# Autodesk Inventor assembly: Bot 1
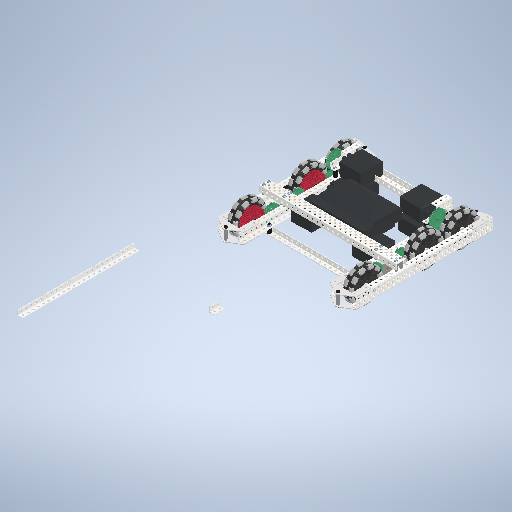
[picture p0: Inventor's stored thumbnail of the model, 512x512]
Saved by Autodesk Inventor 2025.2 (Build 292293000, 293)
## iProperties
Created: 2025-03-17
Part Number: Bot 1
Document SubType Name: Assembly
Designer: Jahan
Author: Jahan
## Documents named in this file (43)
- C:\1629X-7700R-Worlds-Bot\Bot 1\Bot 1.iam
- C:\1629X-7700R-Worlds-Bot\VEX-CAD-Inventor-1.4.2\Structure\C Channel\Aluminum 1x2x1\Alu C 1x2x1x27.ipt
- C:\1629X-7700R-Worlds-Bot\VEX-CAD-Inventor-1.4.2\Structure\C Channel\Aluminum 1x2x1\Alu C 1x2x1x19.ipt
- C:\1629X-7700R-Worlds-Bot\VEX-CAD-Inventor-1.4.2\Motion\Gears\HS Gear.iam
- C:\1629X-7700R-Worlds-Bot\VEX-CAD-Inventor-1.4.2\Motion\Wheels\Omni Wheel\3.25 Omni AS, No Insert.iam
- C:\1629X-7700R-Worlds-Bot\VEX-CAD-Inventor-1.4.2\Motion\Wheels\Omni Wheel.iam
- C:\1629X-7700R-Worlds-Bot\VEX-CAD-Inventor-1.4.2\Motion\Gears\HS Gear\HS 48T Gear, Circle.iam
- C:\1629X-7700R-Worlds-Bot\VEX-CAD-Inventor-1.4.2\Structure\Standoff.ipt
- C:\1629X-7700R-Worlds-Bot\VEX-CAD-Inventor-1.4.2\Structure\Standoff\Standoff .50.ipt
- C:\1629X-7700R-Worlds-Bot\VEX-CAD-Inventor-1.4.2\Motion\Spacers\Washer Teflon.ipt
- C:\1629X-7700R-Worlds-Bot\VEX-CAD-Inventor-1.4.2\Motion\Spacers\Spacer Nylon .375 OD\NSpacer .375 OD x .125.ipt
- C:\1629X-7700R-Worlds-Bot\VEX-CAD-Inventor-1.4.2\Motion\Spacers\Spacer Nylon .375 OD.ipt
- C:\1629X-7700R-Worlds-Bot\VEX-CAD-Inventor-1.4.2\Motion\Spacers\Washer Teflon\TWasher .375 OD x .06250.ipt
- C:\1629X-7700R-Worlds-Bot\VEX-CAD-Inventor-1.4.2\Structure\Hardware\alu_nylock.ipt
- C:\1629X-7700R-Worlds-Bot\VEX-CAD-Inventor-1.4.2\Motion\Gears\LS 36T Gear.ipt
- C:\1629X-7700R-Worlds-Bot\VEX-CAD-Inventor-1.4.2\Motion\Gears\HS Gear\24T HS Gear Cut.iam
- C:\1629X-7700R-Worlds-Bot\VEX-CAD-Inventor-1.4.2\Motion\Shaft LS\Bearing Flat Low Profile.ipt
- C:\1629X-7700R-Worlds-Bot\VEX-CAD-Inventor-1.4.2\Structure\Hardware\Screw Steel - Hex.ipt
- C:\1629X-7700R-Worlds-Bot\VEX-CAD-Inventor-1.4.2\Structure\Hardware\Screw Steel - Hex\SScrew Hex Smooth 1.750.ipt
- C:\1629X-7700R-Worlds-Bot\VEX-CAD-Inventor-1.4.2\Structure\C Channel\Aluminum 1x2x1\Alu C 1x2x1x26.ipt
- C:\1629X-7700R-Worlds-Bot\VEX-CAD-Inventor-1.4.2\Structure\Hardware\Screw Aluminum - Flat Head\AScrew Flat Head Threaded .250.ipt
- C:\1629X-7700R-Worlds-Bot\VEX-CAD-Inventor-1.4.2\Motion\Spacers\Spacer Nylon .375 OD\NSpacer .375 OD x .250.ipt
- C:\1629X-7700R-Worlds-Bot\VEX-CAD-Inventor-1.4.2\Structure\Standoff\Standoff .75.ipt
- C:\1629X-7700R-Worlds-Bot\VEX-CAD-Inventor-1.4.2\Structure\Hardware\Nut Thin Nylock.ipt
- C:\1629X-7700R-Worlds-Bot\VEX-CAD-Inventor-1.4.2\Structure\Hardware\Screw Steel - Star\SScrew Star Smooth .250.ipt
- C:\1629X-7700R-Worlds-Bot\VEX-CAD-Inventor-1.4.2\Structure\Hardware\Screw Steel - Star.ipt
- C:\1629X-7700R-Worlds-Bot\Bot 1\Plastic\backFunnel.ipt
- C:\1629X-7700R-Worlds-Bot\VEX-CAD-Inventor-1.4.2\Structure\Standoff\Standoff 1.00.ipt
- C:\1629X-7700R-Worlds-Bot\VEX-CAD-Inventor-1.4.2\Structure\Angle\Aluminum 1x1\Alu Angle 1x1x19.ipt
- C:\1629X-7700R-Worlds-Bot\VEX-CAD-Inventor-1.4.2\Motion\Spacers\Spacer Nylon .375 OD\NSpacer .375 OD x .500.ipt
- C:\1629X-7700R-Worlds-Bot\VEX-CAD-Inventor-1.4.2\Structure\Hardware\Screw Steel - Star\SScrew Star Smooth .500.ipt
- C:\1629X-7700R-Worlds-Bot\VEX-CAD-Inventor-1.4.2\Electronics\V5 Simple Motor.ipt
- C:\1629X-7700R-Worlds-Bot\VEX-CAD-Inventor-1.4.2\Structure\Hardware\Screw Steel - Star\SScrew Star Smooth .750.ipt
- C:\1629X-7700R-Worlds-Bot\VEX-CAD-Inventor-1.4.2\Structure\Hardware\Screw Nylon - Flat Head\NScrew Flat Head Threaded .250.ipt
- C:\1629X-7700R-Worlds-Bot\VEX-CAD-Inventor-1.4.2\Electronics\V5 Simple Brain.ipt
- C:\1629X-7700R-Worlds-Bot\Bot 1\Plastic\frontFunnel.ipt
- C:\1629X-7700R-Worlds-Bot\VEX-CAD-Inventor-1.4.2\Structure\Angle\Aluminum 1x1\Alu Angle 1x1x2.ipt
- C:\1629X-7700R-Worlds-Bot\VEX-CAD-Inventor-1.4.2\Structure\Angle\Aluminum 1x1\Alu Angle 1x1x23.ipt
- C:\1629X-7700R-Worlds-Bot\VEX-CAD-Inventor-1.4.2\Structure\C Channel\Aluminum 1x2x1\Alu C 1x2x1x3.ipt
- C:\1629X-7700R-Worlds-Bot\VEX-CAD-Inventor-1.4.2\Motion\Spacers\Spacer Nylon .375 OD\NSpacer .375 OD x .375.ipt
- C:\1629X-7700R-Worlds-Bot\VEX-CAD-Inventor-1.4.2\Structure\Angle\Aluminum 1x1\Alu Angle 1x1x5.ipt
- C:\1629X-7700R-Worlds-Bot\VEX-CAD-Inventor-1.4.2\Structure\Hardware\Screw Steel - Star\SScrew Star Smooth 1.000.ipt
- C:\1629X-7700R-Worlds-Bot\VEX-CAD-Inventor-1.4.2\Structure\Hardware\Screw Steel - Star\SScrew Star Smooth .625.ipt
## Components (175 placed, 35 different names)
1. Alu C 1x2x1x26:2 — Insert:72, Insert:73, Insert:74, Insert:105, Insert:106, Insert:130, Insert:132, Insert:141, Insert:142, Insert:143, Insert:144, Insert:151, Insert:152, Insert:163, Mate:8, Flush:1, Insert:164, Insert:165, Insert:169, Insert:181, Insert:186, Insert:206, Insert:210, Insert:213, Insert:228, Insert:229, Insert:257, Insert:264, Insert:274, Insert:275, Insert:276
2. Alu C 1x2x1x26:1 — Insert:5, Insert:6, Insert:75, Insert:76, Insert:77, Insert:107, Insert:108, Insert:125, Insert:126, Insert:139, Insert:140, Insert:145, Insert:146, Insert:147, Insert:148, Insert:149, Insert:150, Insert:182, Insert:184, Insert:204, Insert:211, Insert:212, Insert:225, Insert:227, Insert:233, Insert:241, Insert:242, Insert:243, Insert:252
3. Alu C 1x2x1x27:3 — Insert:5, Insert:6, Insert:7, Insert:8, Insert:9, Insert:10
4. Alu C 1x2x1x27:4 — Insert:7, Insert:8, Insert:52, Insert:58, Insert:65, Insert:81, Insert:82, Insert:83, Insert:127, Insert:128, Insert:170, Insert:171, Insert:172, Insert:173, Insert:183, Insert:203
5. Alu C 1x2x1x27:5 — Insert:9, Insert:10, Insert:25, Insert:31, Insert:39, Insert:43, Insert:44, Insert:45, Insert:46, Insert:78, Insert:79, Insert:80, Insert:129, Insert:131, Insert:166, Insert:167, Insert:168, Insert:180, Insert:205, Insert:208, Insert:209
6. HS 48T Gear, Circle:3 [sub-assembly] — Mate:1
7. 3.25 Omni AS, No Insert:4 [sub-assembly] — Mate:1
8. NSpacer .375 OD x .125:2
9. TWasher .375 OD x .06250:2 — Insert:23
10. alu_nylock:3 — Insert:23, Insert:24
11. Standoff .50:3 — Insert:24, Insert:25
12. HS 48T Gear, Circle:4 [sub-assembly] — Mate:2
13. 3.25 Omni AS, No Insert:5 [sub-assembly] — Mate:2
14. NSpacer .375 OD x .125:3
15. TWasher .375 OD x .06250:3
16. alu_nylock:4
17. Standoff .50:4 — Insert:31
18. HS 48T Gear, Circle:5 [sub-assembly] — Mate:3
19. 3.25 Omni AS, No Insert:6 [sub-assembly] — Mate:3
20. NSpacer .375 OD x .125:4
21. TWasher .375 OD x .06250:4
22. alu_nylock:5
23. Standoff .50:5 — Insert:39
24. Bearing Flat Low Profile:1 — Insert:43, Insert:44
25. Bearing Flat Low Profile:2 — Insert:45, Insert:46
26. HS 48T Gear, Circle:6 [sub-assembly]
27. 3.25 Omni AS, No Insert:7 [sub-assembly]
28. NSpacer .375 OD x .125:6
29. TWasher .375 OD x .06250:5
30. alu_nylock:6
31. Standoff .50:6 — Insert:52
32. HS 48T Gear, Circle:7 [sub-assembly]
33. 3.25 Omni AS, No Insert:8 [sub-assembly]
34. NSpacer .375 OD x .125:7
35. TWasher .375 OD x .06250:6
36. alu_nylock:7
37. Standoff .50:7 — Insert:58
38. HS 48T Gear, Circle:8 [sub-assembly]
39. 3.25 Omni AS, No Insert:9 [sub-assembly]
40. NSpacer .375 OD x .125:8
41. TWasher .375 OD x .06250:7
42. alu_nylock:8
43. Standoff .50:8 — Insert:65
44. SScrew Hex Smooth 1.750:1 — Insert:72
45. SScrew Hex Smooth 1.750:2 — Insert:74
46. SScrew Hex Smooth 1.750:3 — Insert:73
47. SScrew Hex Smooth 1.750:4 — Insert:77
48. SScrew Hex Smooth 1.750:5 — Insert:76
49. SScrew Hex Smooth 1.750:6 — Insert:75
50. AScrew Flat Head Threaded .250:1 — Insert:78
51. AScrew Flat Head Threaded .250:2 — Insert:79
52. AScrew Flat Head Threaded .250:3 — Insert:80
53. AScrew Flat Head Threaded .250:4 — Insert:81
54. AScrew Flat Head Threaded .250:5 — Insert:82
55. AScrew Flat Head Threaded .250:6 — Insert:83
56. Alu C 1x2x1x19:1 — Insert:226, Insert:230, Insert:231, Insert:253, Insert:254, Insert:258
57. Nut Thin Nylock:1 — Insert:105
58. Nut Thin Nylock:2 — Insert:108
59. Nut Thin Nylock:3 — Insert:106
60. Nut Thin Nylock:4 — Insert:107
61. backFunnel:1 — Insert:125, Insert:127, Insert:159
62. backFunnel:2 — Insert:126, Insert:128, Insert:133, Insert:160
63. backFunnel:3 — Insert:129, Insert:130, Insert:161
64. backFunnel:4 — Insert:131, Insert:132, Insert:134, Insert:162
65. Standoff 1.00:17 — Insert:134
66. Standoff 1.00:18 — Insert:133
67. SScrew Star Smooth .500:17 — Insert:141
68. SScrew Star Smooth .500:18 — Insert:146
69. SScrew Star Smooth .500:19 — Insert:144
70. SScrew Star Smooth .500:20 — Insert:145
71. SScrew Star Smooth .500:21 — Insert:143
72. SScrew Star Smooth .500:22 — Insert:139
73. SScrew Star Smooth .500:23 — Insert:140
74. SScrew Star Smooth .500:24 — Insert:142
75. V5 Simple Motor:1 — Insert:147, Insert:148
76. V5 Simple Motor:2 — Insert:149, Insert:150
77. V5 Simple Motor:4 — Insert:151, Insert:152
78. SScrew Star Smooth .750:26 — Insert:189
79. NScrew Flat Head Threaded .250:1 — Insert:159
80. NScrew Flat Head Threaded .250:2 — Insert:160
81. NScrew Flat Head Threaded .250:3 — Insert:162
82. NScrew Flat Head Threaded .250:4 — Insert:161
83. V5 Simple Motor:5 — Insert:163, Mate:8
84. V5 Simple Brain:1
85. frontFunnel:1 — Insert:164, Insert:165, Insert:166, Insert:167, Insert:177
86. frontFunnel:2 — Insert:168, Insert:169, Insert:178, Insert:179
87. frontFunnel:3 — Insert:170, Insert:171, Insert:175
88. frontFunnel:4 — Insert:172, Insert:173, Insert:174, Insert:176
89. Standoff 1.00:19 — Insert:179
90. NScrew Flat Head Threaded .250:5 — Insert:177
91. NScrew Flat Head Threaded .250:6 — Insert:178
92. Standoff 1.00:20 — Insert:176
93. NScrew Flat Head Threaded .250:7 — Insert:174
94. NScrew Flat Head Threaded .250:8 — Insert:175
95. Standoff .75:22 — Mate:16, Insert:209
96. SScrew Star Smooth .250:27 — Mate:14
97. SScrew Star Smooth .250:28 — Mate:15
98. SScrew Star Smooth .250:29 — Mate:12
99. SScrew Star Smooth .250:30 — Mate:11
100. Standoff .75:23 — Mate:10
101. Standoff .75:24 — Mate:9
102. Standoff .75:25 — Insert:197
103. Standoff .75:26 — Insert:196
104. Standoff .75:27 — Insert:193
105. Standoff .75:28 — Insert:192
106. Alu C 1x2x1x27:6 — Insert:192, Insert:193, Insert:194, Insert:195, Insert:196, Insert:197, Insert:198, Insert:199, Mate:9, Mate:10, Mate:11, Mate:12, Mate:14, Mate:15, Mate:16, Insert:207
107. SScrew Star Smooth .250:31 — Insert:198
108. SScrew Star Smooth .250:32 — Insert:199
109. SScrew Star Smooth .250:33 — Insert:195
110. SScrew Star Smooth .250:34 — Insert:194
111. SScrew Star Smooth .250:35 — Insert:181
112. SScrew Star Smooth .250:36 — Insert:180
113. SScrew Star Smooth .250:37 — Insert:182
114. SScrew Star Smooth .250:39 — Insert:183
115. NSpacer .375 OD x .125:16 — Insert:184, Insert:185
116. 24T HS Gear Cut:6 [sub-assembly] — Insert:185
117. 24T HS Gear Cut:7 [sub-assembly] — Insert:187
118. NSpacer .375 OD x .125:17 — Insert:186, Insert:187
119. Nut Thin Nylock:6 — Insert:212
120. NSpacer .375 OD x .500:18 — Insert:190, Insert:211
121. Alu Angle 1x1x19:1 — Insert:188, Insert:189, Insert:190, Insert:191
122. NSpacer .375 OD x .500:19 — Insert:191, Insert:210
123. SScrew Star Smooth .750:40 — Insert:188
124. Alu Angle 1x1x2:1
125. Alu Angle 1x1x23:1
126. SScrew Star Smooth .250:41 — Insert:203
127. SScrew Star Smooth .250:42 — Insert:204
128. Standoff .75:29 — Insert:207, Insert:208
129. SScrew Star Smooth .250:43 — Insert:206
130. SScrew Star Smooth .250:44 — Insert:205
131. Nut Thin Nylock:7 — Insert:213
132. NSpacer .375 OD x .250:22 — Insert:225, Insert:226
133. NSpacer .375 OD x .250:23 — Insert:228, Insert:230
134. NSpacer .375 OD x .250:24 — Insert:227
135. NSpacer .375 OD x .250:25 — Insert:229
136. NSpacer .375 OD x .375:26 — Insert:231, Insert:236
137. NSpacer .375 OD x .375:28 — Insert:234, Insert:235
138. NSpacer .375 OD x .250:29 — Insert:235
139. TWasher .375 OD x .06250:8 — Insert:233, Insert:234
140. LS 36T Gear:9 — Insert:238
141. Alu Angle 1x1x5:1 — Insert:236, Insert:237, Insert:239, Insert:240, Insert:247, Insert:248, Insert:251
142. TWasher .375 OD x .06250:9 — Insert:237, Insert:238
143. SScrew Star Smooth .500:45 — Insert:240
144. SScrew Star Smooth .500:46 — Insert:239
145. LS 36T Gear:10 — Insert:246
146. LS 36T Gear:11 — Insert:245
147. LS 36T Gear:12 — Insert:244
148. TWasher .375 OD x .06250:10 — Insert:241, Insert:244
149. TWasher .375 OD x .06250:11 — Insert:243, Insert:246
150. TWasher .375 OD x .06250:12 — Insert:242, Insert:245
151. V5 Simple Motor:7 — Insert:249, Insert:250
152. Alu C 1x2x1x3:1 — Insert:247, Insert:248, Insert:249, Insert:250
153. SScrew Star Smooth 1.000:49 — Insert:251
154. Nut Thin Nylock:8 — Insert:252
155. SScrew Star Smooth .625:52 — Insert:253
156. SScrew Star Smooth .625:53 — Insert:254
157. NSpacer .375 OD x .375:30
158. NSpacer .375 OD x .250:31 — Insert:259
159. TWasher .375 OD x .06250:13 — Insert:257
160. NSpacer .375 OD x .375:32 — Insert:258, Insert:260
161. V5 Simple Motor:8 — Insert:265, Insert:266
162. Alu C 1x2x1x3:2 — Insert:261, Insert:262, Insert:265, Insert:266
163. Alu Angle 1x1x5:2 — Insert:259, Insert:260, Insert:261, Insert:262, Insert:263, Insert:268, Insert:269, Insert:270
164. SScrew Star Smooth 1.000:54 — Insert:263
165. Nut Thin Nylock:9 — Insert:264
166. LS 36T Gear:13
167. TWasher .375 OD x .06250:14 — Insert:268
168. SScrew Star Smooth .500:55 — Insert:269
169. SScrew Star Smooth .500:56 — Insert:270
170. LS 36T Gear:14
171. TWasher .375 OD x .06250:15 — Insert:275
172. LS 36T Gear:15
173. TWasher .375 OD x .06250:16 — Insert:276
174. LS 36T Gear:16
175. TWasher .375 OD x .06250:17 — Insert:274
## Relationships (204: Insert 189, Mate 14, Flush 1)
- Insert:5: Alu C 1x2x1x26:1 ↔ Alu C 1x2x1x27:3
- Insert:6: Alu C 1x2x1x26:1 ↔ Alu C 1x2x1x27:3
- Insert:7: Alu C 1x2x1x27:3 ↔ Alu C 1x2x1x27:4
- Insert:8: Alu C 1x2x1x27:3 ↔ Alu C 1x2x1x27:4
- Insert:9: Alu C 1x2x1x27:3 ↔ Alu C 1x2x1x27:5
- Insert:10: Alu C 1x2x1x27:3 ↔ Alu C 1x2x1x27:5
- [Insert]: HS 48T Gear, Circle:3 ↔ 3.25 Omni AS, No Insert:4
- [Insert]: HS 48T Gear, Circle:3 ↔ NSpacer .375 OD x .125:2
- [Insert]: 3.25 Omni AS, No Insert:4 ↔ TWasher .375 OD x .06250:2
- Insert:23: TWasher .375 OD x .06250:2 ↔ alu_nylock:3
- Insert:24: alu_nylock:3 ↔ Standoff .50:3
- Insert:25: Alu C 1x2x1x27:5 ↔ Standoff .50:3
- [Insert]: HS 48T Gear, Circle:4 ↔ 3.25 Omni AS, No Insert:5
- [Insert]: HS 48T Gear, Circle:4 ↔ NSpacer .375 OD x .125:3
- [Insert]: 3.25 Omni AS, No Insert:5 ↔ TWasher .375 OD x .06250:3
- [Insert]: TWasher .375 OD x .06250:3 ↔ alu_nylock:4
- [Insert]: alu_nylock:4 ↔ Standoff .50:4
- Insert:31: Alu C 1x2x1x27:5 ↔ Standoff .50:4
- [Insert]: HS 48T Gear, Circle:5 ↔ 3.25 Omni AS, No Insert:6
- [Insert]: HS 48T Gear, Circle:5 ↔ NSpacer .375 OD x .125:4
- [Insert]: 3.25 Omni AS, No Insert:6 ↔ TWasher .375 OD x .06250:4
- [Insert]: TWasher .375 OD x .06250:4 ↔ alu_nylock:5
- [Insert]: alu_nylock:5 ↔ Standoff .50:5
- Insert:39: Alu C 1x2x1x27:5 ↔ Standoff .50:5
- Mate:1: HS 48T Gear, Circle:3 ↔ 3.25 Omni AS, No Insert:4
- Mate:2: HS 48T Gear, Circle:4 ↔ 3.25 Omni AS, No Insert:5
- Mate:3: HS 48T Gear, Circle:5 ↔ 3.25 Omni AS, No Insert:6
- Insert:43: Alu C 1x2x1x27:5 ↔ Bearing Flat Low Profile:1
- Insert:44: Alu C 1x2x1x27:5 ↔ Bearing Flat Low Profile:1
- Insert:45: Alu C 1x2x1x27:5 ↔ Bearing Flat Low Profile:2
- Insert:46: Alu C 1x2x1x27:5 ↔ Bearing Flat Low Profile:2
- [Insert]: HS 48T Gear, Circle:6 ↔ 3.25 Omni AS, No Insert:7
- [Insert]: HS 48T Gear, Circle:6 ↔ NSpacer .375 OD x .125:6
- [Insert]: 3.25 Omni AS, No Insert:7 ↔ TWasher .375 OD x .06250:5
- [Insert]: TWasher .375 OD x .06250:5 ↔ alu_nylock:6
- [Insert]: alu_nylock:6 ↔ Standoff .50:6
- [Mate]: HS 48T Gear, Circle:6 ↔ 3.25 Omni AS, No Insert:7
- Insert:52: Alu C 1x2x1x27:4 ↔ Standoff .50:6
- [Insert]: HS 48T Gear, Circle:7 ↔ 3.25 Omni AS, No Insert:8
- [Insert]: HS 48T Gear, Circle:7 ↔ NSpacer .375 OD x .125:7
- [Insert]: 3.25 Omni AS, No Insert:8 ↔ TWasher .375 OD x .06250:6
- [Insert]: TWasher .375 OD x .06250:6 ↔ alu_nylock:7
- [Insert]: alu_nylock:7 ↔ Standoff .50:7
- [Mate]: HS 48T Gear, Circle:7 ↔ 3.25 Omni AS, No Insert:8
- Insert:58: Alu C 1x2x1x27:4 ↔ Standoff .50:7
- [Insert]: HS 48T Gear, Circle:8 ↔ 3.25 Omni AS, No Insert:9
- [Insert]: HS 48T Gear, Circle:8 ↔ NSpacer .375 OD x .125:8
- [Insert]: 3.25 Omni AS, No Insert:9 ↔ TWasher .375 OD x .06250:7
- [Insert]: TWasher .375 OD x .06250:7 ↔ alu_nylock:8
- [Insert]: alu_nylock:8 ↔ Standoff .50:8
- [Mate]: HS 48T Gear, Circle:8 ↔ 3.25 Omni AS, No Insert:9
- Insert:65: Alu C 1x2x1x27:4 ↔ Standoff .50:8
- Insert:72: Alu C 1x2x1x26:2 ↔ SScrew Hex Smooth 1.750:1
- Insert:73: Alu C 1x2x1x26:2 ↔ SScrew Hex Smooth 1.750:3
- Insert:74: Alu C 1x2x1x26:2 ↔ SScrew Hex Smooth 1.750:2
- Insert:75: Alu C 1x2x1x26:1 ↔ SScrew Hex Smooth 1.750:6
- Insert:76: Alu C 1x2x1x26:1 ↔ SScrew Hex Smooth 1.750:5
- Insert:77: Alu C 1x2x1x26:1 ↔ SScrew Hex Smooth 1.750:4
- Insert:78: Alu C 1x2x1x27:5 ↔ AScrew Flat Head Threaded .250:1
- Insert:79: Alu C 1x2x1x27:5 ↔ AScrew Flat Head Threaded .250:2
- Insert:80: Alu C 1x2x1x27:5 ↔ AScrew Flat Head Threaded .250:3
- Insert:81: Alu C 1x2x1x27:4 ↔ AScrew Flat Head Threaded .250:4
- Insert:82: Alu C 1x2x1x27:4 ↔ AScrew Flat Head Threaded .250:5
- Insert:83: Alu C 1x2x1x27:4 ↔ AScrew Flat Head Threaded .250:6
- Insert:105: Alu C 1x2x1x26:2 ↔ Nut Thin Nylock:1
- Insert:106: Alu C 1x2x1x26:2 ↔ Nut Thin Nylock:3
- Insert:107: Alu C 1x2x1x26:1 ↔ Nut Thin Nylock:4
- Insert:108: Alu C 1x2x1x26:1 ↔ Nut Thin Nylock:2
- Insert:125: Alu C 1x2x1x26:1 ↔ backFunnel:1
- Insert:126: Alu C 1x2x1x26:1 ↔ backFunnel:2
- Insert:127: Alu C 1x2x1x27:4 ↔ backFunnel:1
- Insert:128: Alu C 1x2x1x27:4 ↔ backFunnel:2
- Insert:129: Alu C 1x2x1x27:5 ↔ backFunnel:3
- Insert:130: Alu C 1x2x1x26:2 ↔ backFunnel:3
- Insert:131: Alu C 1x2x1x27:5 ↔ backFunnel:4
- Insert:132: Alu C 1x2x1x26:2 ↔ backFunnel:4
- Insert:133: backFunnel:2 ↔ Standoff 1.00:18
- Insert:134: backFunnel:4 ↔ Standoff 1.00:17
- Insert:139: Alu C 1x2x1x26:1 ↔ SScrew Star Smooth .500:22
- Insert:140: Alu C 1x2x1x26:1 ↔ SScrew Star Smooth .500:23
- Insert:141: Alu C 1x2x1x26:2 ↔ SScrew Star Smooth .500:17
- Insert:142: Alu C 1x2x1x26:2 ↔ SScrew Star Smooth .500:24
- Insert:143: Alu C 1x2x1x26:2 ↔ SScrew Star Smooth .500:21
- Insert:144: Alu C 1x2x1x26:2 ↔ SScrew Star Smooth .500:19
- Insert:145: Alu C 1x2x1x26:1 ↔ SScrew Star Smooth .500:20
- Insert:146: Alu C 1x2x1x26:1 ↔ SScrew Star Smooth .500:18
- Insert:147: Alu C 1x2x1x26:1 ↔ V5 Simple Motor:1
- Insert:148: Alu C 1x2x1x26:1 ↔ V5 Simple Motor:1
- Insert:149: Alu C 1x2x1x26:1 ↔ V5 Simple Motor:2
- Insert:150: Alu C 1x2x1x26:1 ↔ V5 Simple Motor:2
- Insert:151: Alu C 1x2x1x26:2 ↔ V5 Simple Motor:4
- Insert:152: Alu C 1x2x1x26:2 ↔ V5 Simple Motor:4
- Insert:159: backFunnel:1 ↔ NScrew Flat Head Threaded .250:1
- Insert:160: backFunnel:2 ↔ NScrew Flat Head Threaded .250:2
- Insert:161: backFunnel:3 ↔ NScrew Flat Head Threaded .250:4
- Insert:162: backFunnel:4 ↔ NScrew Flat Head Threaded .250:3
- Insert:163: Alu C 1x2x1x26:2 ↔ V5 Simple Motor:5
- Mate:8: Alu C 1x2x1x26:2 ↔ V5 Simple Motor:5
- Flush:1: Alu C 1x2x1x26:2
- Insert:164: Alu C 1x2x1x26:2 ↔ frontFunnel:1
- Insert:165: Alu C 1x2x1x26:2 ↔ frontFunnel:1
- Insert:166: Alu C 1x2x1x27:5 ↔ frontFunnel:1
- Insert:167: Alu C 1x2x1x27:5 ↔ frontFunnel:1
- Insert:168: Alu C 1x2x1x27:5 ↔ frontFunnel:2
- Insert:169: Alu C 1x2x1x26:2 ↔ frontFunnel:2
- Insert:170: Alu C 1x2x1x27:4 ↔ frontFunnel:3
- Insert:171: Alu C 1x2x1x27:4 ↔ frontFunnel:3
- Insert:172: Alu C 1x2x1x27:4 ↔ frontFunnel:4
- Insert:173: Alu C 1x2x1x27:4 ↔ frontFunnel:4
- Insert:174: frontFunnel:4 ↔ NScrew Flat Head Threaded .250:7
- Insert:175: frontFunnel:3 ↔ NScrew Flat Head Threaded .250:8
- Insert:176: frontFunnel:4 ↔ Standoff 1.00:20
- Insert:177: frontFunnel:1 ↔ NScrew Flat Head Threaded .250:5
- Insert:178: frontFunnel:2 ↔ NScrew Flat Head Threaded .250:6
- Insert:179: frontFunnel:2 ↔ Standoff 1.00:19
- Insert:180: Alu C 1x2x1x27:5 ↔ SScrew Star Smooth .250:36
- Insert:181: Alu C 1x2x1x26:2 ↔ SScrew Star Smooth .250:35
- Insert:182: Alu C 1x2x1x26:1 ↔ SScrew Star Smooth .250:37
- Insert:183: Alu C 1x2x1x27:4 ↔ SScrew Star Smooth .250:39
- Insert:184: Alu C 1x2x1x26:1 ↔ NSpacer .375 OD x .125:16
- Insert:185: NSpacer .375 OD x .125:16 ↔ 24T HS Gear Cut:6
- Insert:186: Alu C 1x2x1x26:2 ↔ NSpacer .375 OD x .125:17
- Insert:187: 24T HS Gear Cut:7 ↔ NSpacer .375 OD x .125:17
- Insert:188: Alu Angle 1x1x19:1 ↔ SScrew Star Smooth .750:40
- Insert:189: SScrew Star Smooth .750:26 ↔ Alu Angle 1x1x19:1
- Insert:190: NSpacer .375 OD x .500:18 ↔ Alu Angle 1x1x19:1
- Insert:191: Alu Angle 1x1x19:1 ↔ NSpacer .375 OD x .500:19
- Insert:192: Standoff .75:28 ↔ Alu C 1x2x1x27:6
- Insert:193: Standoff .75:27 ↔ Alu C 1x2x1x27:6
- Insert:194: Alu C 1x2x1x27:6 ↔ SScrew Star Smooth .250:34
- Insert:195: Alu C 1x2x1x27:6 ↔ SScrew Star Smooth .250:33
- Insert:196: Standoff .75:26 ↔ Alu C 1x2x1x27:6
- Insert:197: Standoff .75:25 ↔ Alu C 1x2x1x27:6
- Insert:198: Alu C 1x2x1x27:6 ↔ SScrew Star Smooth .250:31
- Insert:199: Alu C 1x2x1x27:6 ↔ SScrew Star Smooth .250:32
- Mate:9: Standoff .75:24 ↔ Alu C 1x2x1x27:6
- Mate:10: Standoff .75:23 ↔ Alu C 1x2x1x27:6
- Mate:11: SScrew Star Smooth .250:30 ↔ Alu C 1x2x1x27:6
- Mate:12: SScrew Star Smooth .250:29 ↔ Alu C 1x2x1x27:6
- Mate:14: SScrew Star Smooth .250:27 ↔ Alu C 1x2x1x27:6
- Mate:15: SScrew Star Smooth .250:28 ↔ Alu C 1x2x1x27:6
- Mate:16: Standoff .75:22 ↔ Alu C 1x2x1x27:6
- Insert:203: Alu C 1x2x1x27:4 ↔ SScrew Star Smooth .250:41
- Insert:204: Alu C 1x2x1x26:1 ↔ SScrew Star Smooth .250:42
- Insert:205: Alu C 1x2x1x27:5 ↔ SScrew Star Smooth .250:44
- Insert:206: Alu C 1x2x1x26:2 ↔ SScrew Star Smooth .250:43
- Insert:207: Alu C 1x2x1x27:6 ↔ Standoff .75:29
- Insert:208: Alu C 1x2x1x27:5 ↔ Standoff .75:29
- Insert:209: Alu C 1x2x1x27:5 ↔ Standoff .75:22
- Insert:210: Alu C 1x2x1x26:2 ↔ NSpacer .375 OD x .500:19
- Insert:211: Alu C 1x2x1x26:1 ↔ NSpacer .375 OD x .500:18
- Insert:212: Alu C 1x2x1x26:1 ↔ Nut Thin Nylock:6
- Insert:213: Alu C 1x2x1x26:2 ↔ Nut Thin Nylock:7
- Insert:225: Alu C 1x2x1x26:1 ↔ NSpacer .375 OD x .250:22
- Insert:226: Alu C 1x2x1x19:1 ↔ NSpacer .375 OD x .250:22
- Insert:227: Alu C 1x2x1x26:1 ↔ NSpacer .375 OD x .250:24
- Insert:228: Alu C 1x2x1x26:2 ↔ NSpacer .375 OD x .250:23
- Insert:229: Alu C 1x2x1x26:2 ↔ NSpacer .375 OD x .250:25
- Insert:230: Alu C 1x2x1x19:1 ↔ NSpacer .375 OD x .250:23
- Insert:231: Alu C 1x2x1x19:1 ↔ NSpacer .375 OD x .375:26
- Insert:233: Alu C 1x2x1x26:1 ↔ TWasher .375 OD x .06250:8
- Insert:234: NSpacer .375 OD x .375:28 ↔ TWasher .375 OD x .06250:8
- Insert:235: NSpacer .375 OD x .375:28 ↔ NSpacer .375 OD x .250:29
- Insert:236: NSpacer .375 OD x .375:26 ↔ Alu Angle 1x1x5:1
- Insert:237: Alu Angle 1x1x5:1 ↔ TWasher .375 OD x .06250:9
- Insert:238: LS 36T Gear:9 ↔ TWasher .375 OD x .06250:9
- Insert:239: Alu Angle 1x1x5:1 ↔ SScrew Star Smooth .500:46
- Insert:240: Alu Angle 1x1x5:1 ↔ SScrew Star Smooth .500:45
- Insert:241: Alu C 1x2x1x26:1 ↔ TWasher .375 OD x .06250:10
- Insert:242: Alu C 1x2x1x26:1 ↔ TWasher .375 OD x .06250:12
- Insert:243: Alu C 1x2x1x26:1 ↔ TWasher .375 OD x .06250:11
- Insert:244: LS 36T Gear:12 ↔ TWasher .375 OD x .06250:10
- Insert:245: LS 36T Gear:11 ↔ TWasher .375 OD x .06250:12
- Insert:246: LS 36T Gear:10 ↔ TWasher .375 OD x .06250:11
- Insert:247: Alu Angle 1x1x5:1 ↔ Alu C 1x2x1x3:1
- Insert:248: Alu Angle 1x1x5:1 ↔ Alu C 1x2x1x3:1
- Insert:249: V5 Simple Motor:7 ↔ Alu C 1x2x1x3:1
- Insert:250: V5 Simple Motor:7 ↔ Alu C 1x2x1x3:1
- Insert:251: Alu Angle 1x1x5:1 ↔ SScrew Star Smooth 1.000:49
- Insert:252: Alu C 1x2x1x26:1 ↔ Nut Thin Nylock:8
- Insert:253: Alu C 1x2x1x19:1 ↔ SScrew Star Smooth .625:52
- Insert:254: Alu C 1x2x1x19:1 ↔ SScrew Star Smooth .625:53
- [Insert]: NSpacer .375 OD x .375:30 ↔ TWasher .375 OD x .06250:13
- [Insert]: NSpacer .375 OD x .375:30 ↔ NSpacer .375 OD x .250:31
- Insert:257: Alu C 1x2x1x26:2 ↔ TWasher .375 OD x .06250:13
- Insert:258: Alu C 1x2x1x19:1 ↔ NSpacer .375 OD x .375:32
- Insert:259: NSpacer .375 OD x .250:31 ↔ Alu Angle 1x1x5:2
- Insert:260: NSpacer .375 OD x .375:32 ↔ Alu Angle 1x1x5:2
- Insert:261: Alu C 1x2x1x3:2 ↔ Alu Angle 1x1x5:2
- Insert:262: Alu C 1x2x1x3:2 ↔ Alu Angle 1x1x5:2
- Insert:263: Alu Angle 1x1x5:2 ↔ SScrew Star Smooth 1.000:54
- Insert:264: Alu C 1x2x1x26:2 ↔ Nut Thin Nylock:9
- Insert:265: V5 Simple Motor:8 ↔ Alu C 1x2x1x3:2
- Insert:266: V5 Simple Motor:8 ↔ Alu C 1x2x1x3:2
- [Insert]: LS 36T Gear:13 ↔ TWasher .375 OD x .06250:14
- Insert:268: Alu Angle 1x1x5:2 ↔ TWasher .375 OD x .06250:14
- Insert:269: Alu Angle 1x1x5:2 ↔ SScrew Star Smooth .500:55
- Insert:270: Alu Angle 1x1x5:2 ↔ SScrew Star Smooth .500:56
- [Insert]: LS 36T Gear:14 ↔ TWasher .375 OD x .06250:15
- [Insert]: LS 36T Gear:15 ↔ TWasher .375 OD x .06250:16
- [Insert]: LS 36T Gear:16 ↔ TWasher .375 OD x .06250:17
- Insert:274: Alu C 1x2x1x26:2 ↔ TWasher .375 OD x .06250:17
- Insert:275: Alu C 1x2x1x26:2 ↔ TWasher .375 OD x .06250:15
- Insert:276: Alu C 1x2x1x26:2 ↔ TWasher .375 OD x .06250:16
## Named parameters: d122_d116 = 0 mm, d123_d117 = 0 mm, d124_d119 = 0 mm, d129_d122_d116 = 0 mm, d130_d123_d117 = 0 mm, d131_d124_d119 = 0 mm, d132_d126 = 0 mm, d133_d127 = 0 mm, d144_d129_d122_d116 = 0 mm, d145_d130_d123_d117 = 0 mm, d146_d131_d124_d119 = 0 mm, d147_d132_d126 = 0 mm, d148_d133_d127 = 0 mm, d162_d127 = 0 mm, d163_d153 = 0 mm, d164_d122_d116 = 0 mm, d165_d123_d117 = 0 mm, d166_d124_d119 = 0 mm, d167_d126 = 0 mm, d169_d127 = 0 mm, d170_d153 = 0 mm, d171_d122_d116 = 0 mm, d172_d123_d117 = 0 mm, d173_d124_d119 = 0 mm, d174_d126 = 0 mm, d177_d169_d127 = 0 mm, d178_d170_d153 = 0 mm, d179_d171_d122_d116 = 0 mm, d180_d172_d123_d117 = 0 mm, d181_d173_d124_d119 = 0 mm, d182_d174_d126 = 0 mm, d430_d409 = 0 mm, d431_d410 = 0 mm, d442_d413 = 0 mm, d446_d442_d413 = 0 mm, d447_d442_d413 = 0 mm, d448_d442_d413 = 0 mm
